# Autodesk Inventor assembly: Rainbovv Reincarnation
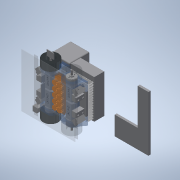
[picture p0: Inventor's stored thumbnail of the model, 180x180]
Saved by Autodesk Inventor 2020 (Build 240168000, 168)
## iProperties
Created: 2019-01-30
Part Number: Rainbovv Reincarnation
Material: Ogólny
Document SubType Name: Assembly
Designer: atmat
Author: atmat
## Documents named in this file (14)
- C:\Users\atmat\Documents\1.Projects\1.Roboty\1.Rainbow\1.Reincarnation\Czesci\Ver 1\Rainbovv Reincarnation.iam
- C:\Users\atmat\Documents\1.Projects\1.Roboty\1.Rainbow\1.Reincarnation\Czesci\Ver 1\Motor.ipt
- C:\Users\atmat\Documents\1.Projects\1.Roboty\1.Rainbow\1.Reincarnation\Czesci\Ver 1\Wheel.ipt
- C:\Users\atmat\Documents\1.Projects\1.Roboty\1.Rainbow\1.Reincarnation\Czesci\Ver 1\Sharp.ipt
- C:\Users\atmat\Documents\1.Projects\1.Roboty\1.Rainbow\1.Reincarnation\Czesci\Ver 1\Peltier.ipt
- C:\Users\atmat\Documents\1.Projects\1.Roboty\1.Rainbow\1.Reincarnation\Czesci\Ver 1\pcb.ipt
- C:\Users\atmat\Documents\1.Projects\1.Roboty\1.Rainbow\1.Reincarnation\Czesci\Ver 1\Radiator.ipt
- C:\Users\atmat\Documents\1.Projects\1.Roboty\1.Rainbow\1.Reincarnation\Czesci\Ver 1\pcb_bottom.ipt
- C:\Users\atmat\Documents\1.Projects\1.Roboty\1.Rainbow\1.Reincarnation\Czesci\Ver 1\UberDriver.ipt
- C:\Users\atmat\Documents\1.Projects\1.Roboty\1.Rainbow\1.Reincarnation\Czesci\Ver 1\vl.ipt
- C:\Users\atmat\Documents\1.Projects\1.Roboty\1.Rainbow\1.Reincarnation\Czesci\Ver 1\Holder.ipt
- C:\Users\atmat\Documents\1.Projects\1.Roboty\Kryptonim Bunny\Invertor\Bateria.ipt
- C:\Users\atmat\Documents\1.Projects\1.Roboty\1.Rainbow\1.Reincarnation\Czesci\Ver 2\Bateria_22V2_Rozlozona.ipt
- C:\Users\atmat\Documents\1.Projects\1.Roboty\1.Rainbow\1.Reincarnation\Czesci\S5_Mainboard.ipt
## Components (29 placed, 13 different names)
1. Motor:1 — Równoległy:1, Równoległy:2, Równoległy:3, Zestawiający:1, Zestawiający:2, Równoległy:4, Równoległy:6, Wstaw:4
2. Motor:2 — Równoległy:2, Zestawiający:2, Równoległy:6, Wstaw:2, Równoległy:14, Zestawiający:15, Zestawiający:16, Zestawiający:26
3. Motor:3 — Równoległy:1, Zestawiający:1, Równoległy:5, Wstaw:1, Zestawiający:20, Zestawiający:26
4. Motor:4 — Równoległy:3, Równoległy:4, Równoległy:5, Wstaw:3, Zestawiający:8, Zestawiający:17, Zestawiający:28
5. Wheel:1 — Wstaw:2
6. Wheel:2 — Wstaw:1, Zestawiający:9
7. Wheel:3 — Wstaw:3, Styczny:1, Zestawiający:10, Styczny:2, Równoległy:23, Zestawiający:22, Zestawiający:24
8. Wheel:4 — Wstaw:4, Styczny:1, Zestawiający:19, Styczny:3
9. Sharp:1 — Równoległy:7, Równoległy:10, Kąt:1, Zestawiający:5, Zestawiający:6, Równoległy:20, Równoległy:21
10. Sharp:2 — Równoległy:13, Kąt:1, Zestawiający:5, Zestawiający:6, Zestawiający:9
11. Sharp:3 — Równoległy:12, Kąt:2, Zestawiający:3, Zestawiający:4, Równoległy:14, Zestawiający:10
12. Sharp:4 — Równoległy:7, Równoległy:10, Równoległy:12, Równoległy:13, Kąt:2, Zestawiający:3, Zestawiający:4, Zestawiający:8, Równoległy:19, Zestawiający:23
13. Sharp:5 — Równoległy:19
14. Sharp:6
15. Sharp:7
16. Sharp:8 — Równoległy:20, Równoległy:21, Zestawiający:15, Równoległy:29, Zestawiający:30
17. Peltier:1 — Zestawiający:16, Zestawiający:18, Równoległy:22, Zestawiający:19, Zestawiający:27, Zestawiający:33, Równoległy:33
18. Peltier:2 — Zestawiający:17, Zestawiający:18, Równoległy:22, Zestawiający:20, Zestawiający:21, Równoległy:24
19. pcb:1 — Styczny:2, Styczny:3, Równoległy:23, Równoległy:25, Zestawiający:25, Równoległy:27
20. Radiator:1 — Zestawiający:21, Zestawiający:22, Równoległy:24, Równoległy:25, Równoległy:26, Równoległy:28, Zestawiający:32, Równoległy:32, Równoległy:34
21. pcb_bottom:1 — Zestawiający:23, Równoległy:26, Zestawiający:24, Zestawiający:29, Zestawiający:31, Równoległy:30, Równoległy:31
22. UberDriver:1 — Równoległy:28, Zestawiający:27, Zestawiający:28
23. vl:1 — Zestawiający:29, Równoległy:29, Zestawiający:30
24. vl:2
25. Sharp:9 — Zestawiający:31, Równoległy:30, Równoległy:31
26. Holder:1 — Zestawiający:32, Zestawiający:33, Równoległy:32
27. Bateria:1 — Równoległy:33, Równoległy:34
28. Bateria_22V2_Rozlozona:1
29. S5_Mainboard:1
## Relationships (74: Mate 32, Flush 31, Insert 4, Angle 4, Tangent 3)
- Równoległy:1 [Flush]: Motor:1 ↔ Motor:3
- Równoległy:2 [Flush]: Motor:1 ↔ Motor:2
- Równoległy:3 [Flush]: Motor:1 ↔ Motor:4
- Zestawiający:1 [Mate] (3.22 mm): Motor:1 ↔ Motor:3
- Zestawiający:2 [Mate] (3.22 mm): Motor:1 ↔ Motor:2
- Równoległy:4 [Flush]: Motor:1 ↔ Motor:4
- Równoległy:5 [Flush]: Motor:3 ↔ Motor:4
- Równoległy:6 [Flush]: Motor:1 ↔ Motor:2
- Wstaw:1 [Insert]: Motor:3 ↔ Wheel:2
- Wstaw:2 [Insert]: Motor:2 ↔ Wheel:1
- Wstaw:3 [Insert]: Motor:4 ↔ Wheel:3
- Wstaw:4 [Insert]: Motor:1 ↔ Wheel:4
- Styczny:1 [Tangent] (18 mm): Wheel:3 ↔ Wheel:4
- Równoległy:7 [Flush]: Sharp:1 ↔ Sharp:4
- Równoległy:10 [Flush]: Sharp:1 ↔ Sharp:4
- Równoległy:12 [Flush]: Sharp:3 ↔ Sharp:4
- Równoległy:13 [Flush]: Sharp:2 ↔ Sharp:4
- Kąt:1 [Angle] (225 deg): Sharp:1 ↔ Sharp:2
- Kąt:2 [Angle] (135 deg): Sharp:3 ↔ Sharp:4
- Zestawiający:3 [Mate] (1 mm): Sharp:3 ↔ Sharp:4
- Zestawiający:4 [Mate]: Sharp:3 ↔ Sharp:4
- Zestawiający:5 [Mate] (1 mm): Sharp:1 ↔ Sharp:2
- Zestawiający:6 [Mate]: Sharp:1 ↔ Sharp:2
- Równoległy:14 [Flush]: Motor:2 ↔ Sharp:3
- Zestawiający:8 [Mate] (8.65 mm): Motor:4 ↔ Sharp:4
- Zestawiający:9 [Mate] (5 mm): Wheel:2 ↔ Sharp:2
- Zestawiający:10 [Mate] (5 mm): Wheel:3 ↔ Sharp:3
- [Flush]: Sharp:5 ↔ Sharp:8
- [Flush]: Sharp:5 ↔ Sharp:8
- [Flush]: Sharp:7 ↔ Sharp:8
- [Flush]: Sharp:6 ↔ Sharp:8
- [Angle] (225 deg): Sharp:5 ↔ Sharp:6
- [Angle] (135 deg): Sharp:7 ↔ Sharp:8
- [Mate] (1 mm): Sharp:7 ↔ Sharp:8
- [Mate]: Sharp:7 ↔ Sharp:8
- [Mate] (1 mm): Sharp:5 ↔ Sharp:6
- [Mate]: Sharp:5 ↔ Sharp:6
- Równoległy:19 [Flush]: Sharp:4 ↔ Sharp:5
- Równoległy:20 [Flush]: Sharp:1 ↔ Sharp:8
- Równoległy:21 [Flush]: Sharp:1 ↔ Sharp:8
- Zestawiający:15 [Mate] (8.65 mm): Motor:2 ↔ Sharp:8
- Zestawiający:16 [Mate]: Motor:2 ↔ Peltier:1
- Zestawiający:17 [Mate]: Motor:4 ↔ Peltier:2
- Zestawiający:18 [Mate] (1 mm): Peltier:1 ↔ Peltier:2
- Równoległy:22 [Flush]: Peltier:1 ↔ Peltier:2
- Zestawiający:19 [Mate] (15.57 mm): Wheel:4 ↔ Peltier:1
- Zestawiający:20 [Mate] (-19.15 mm): Motor:3 ↔ Peltier:2
- Styczny:2 [Tangent]: Wheel:3 ↔ pcb:1
- Styczny:3 [Tangent]: Wheel:4 ↔ pcb:1
- Równoległy:23 [Flush] (-1.23 mm): Wheel:3 ↔ pcb:1
- Zestawiający:21 [Mate]: Peltier:2 ↔ Radiator:1
- Zestawiający:22 [Mate] (5.57 mm): Wheel:3 ↔ Radiator:1
- Równoległy:24 [Flush]: Peltier:2 ↔ Radiator:1
- Równoległy:25 [Flush]: pcb:1 ↔ Radiator:1
- Zestawiający:23 [Mate]: Sharp:4 ↔ pcb_bottom:1
- Równoległy:26 [Flush]: Radiator:1 ↔ pcb_bottom:1
- Zestawiający:24 [Mate] (7.57 mm): Wheel:3 ↔ pcb_bottom:1
- Zestawiający:25 [Mate]: pcb:1
- Równoległy:27 [Flush]: pcb:1
- Zestawiający:26 [Mate] (39.3 mm): Motor:2 ↔ Motor:3
- Równoległy:28 [Flush] (2.06 mm): Radiator:1 ↔ UberDriver:1
- Zestawiający:27 [Mate]: Peltier:1 ↔ UberDriver:1
- Zestawiający:28 [Mate] (10.285 mm): Motor:4 ↔ UberDriver:1
- Zestawiający:29 [Mate]: pcb_bottom:1 ↔ vl:1
- Równoległy:29 [Flush]: Sharp:8 ↔ vl:1
- Zestawiający:30 [Mate]: Sharp:8 ↔ vl:1
- Zestawiający:31 [Mate]: pcb_bottom:1 ↔ Sharp:9
- Równoległy:30 [Flush]: pcb_bottom:1 ↔ Sharp:9
- Równoległy:31 [Flush] (3 mm): pcb_bottom:1 ↔ Sharp:9
- Zestawiający:32 [Mate]: Radiator:1 ↔ Holder:1
- Zestawiający:33 [Mate]: Peltier:1 ↔ Holder:1
- Równoległy:32 [Flush]: Radiator:1 ↔ Holder:1
- Równoległy:33 [Flush] (15 mm): Peltier:1 ↔ Bateria:1
- Równoległy:34 [Flush]: Radiator:1 ↔ Bateria:1
## Named parameters: d32_d20 = 0 mm, d33_d21 = 225 deg, d34_d22 = 135 deg, d35_d23 = 1 mm, d36_d24 = 0 mm, d37_d25 = 1 mm, d38_d26 = 0 mm, d39_d13 = 0 mm, d40_d16 = 0 mm, d41_d19 = 0 mm
